# Autodesk Inventor assembly: Cangrejo-Sin-Reductores
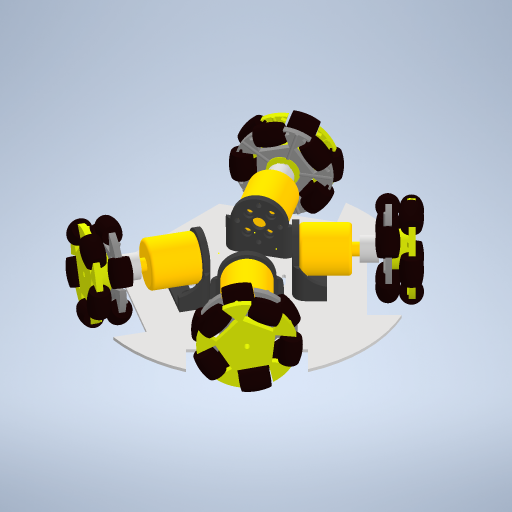
[picture p0: Inventor's stored thumbnail of the model, 512x512]
Saved by Autodesk Inventor 2024 (Build 280153000, 153)
## iProperties
Created: 2023-11-21
Part Number: Cangrejo-Sin-Reductores
Document SubType Name: Assembly
Designer: felip
Author: felip
## Documents named in this file (5)
- C:\Users\felip\Downloads\Gemelo Digital V2\Cangrejo-Sin-Reductores.iam
- C:\Users\felip\Downloads\Gemelo Digital V2\BaseV7.ipt
- C:\Users\felip\Downloads\Gemelo Digital V2\Motor-Soporte-Montaje.iam
- C:\Users\felip\Downloads\Gemelo Digital V2\OMNIWHEELV4.iam
- C:\Users\felip\Downloads\Gemelo Digital V2\Pseudo-SunGear.ipt
## Components (13 placed, 4 different names)
1. BaseV7:1 — Rotational:1, Rotational:2, Rotational:3, Rotational:4, Rotational:12, Rotational:13, Rotational:15, Rotational:16
2. Motor-Soporte-Montaje:1 [sub-assembly] — Rotational:1, Rotational:2, Rotational:7
3. OMNIWHEELV4:1 [sub-assembly] — Rotational:14
4. Pseudo-SunGear:2 — Rotational:7, Rotational:17
5. Pseudo-SunGear:4 — Rotational:8, Rotational:14
6. Motor-Soporte-Montaje:2 [sub-assembly] — Rotational:3, Rotational:4, Rotational:8
7. OMNIWHEELV4:2 [sub-assembly] — Rotational:9
8. OMNIWHEELV4:4 [sub-assembly] — Rotational:17
9. Pseudo-SunGear:5 — Rotational:9
10. Motor-Soporte-Montaje:4 [sub-assembly] — Rotational:15, Rotational:16
11. OMNIWHEELV4:5 [sub-assembly]
12. Pseudo-SunGear:6
13. Motor-Soporte-Montaje:5 [sub-assembly] — Rotational:12, Rotational:13
## Relationships (16: RevoluteJoint 16)
- Rotational:1 [RevoluteJoint]: BaseV7:1 ↔ Motor-Soporte-Montaje:1
- Rotational:2 [RevoluteJoint]: BaseV7:1 ↔ Motor-Soporte-Montaje:1
- Rotational:3 [RevoluteJoint]: BaseV7:1 ↔ Motor-Soporte-Montaje:2
- Rotational:4 [RevoluteJoint]: BaseV7:1 ↔ Motor-Soporte-Montaje:2
- [RevoluteJoint]: Pseudo-SunGear:5 ↔ Motor-Soporte-Montaje:4
- Rotational:7 [RevoluteJoint]: Motor-Soporte-Montaje:1 ↔ Pseudo-SunGear:2
- Rotational:8 [RevoluteJoint]: Pseudo-SunGear:4 ↔ Motor-Soporte-Montaje:2
- Rotational:9 [RevoluteJoint]: OMNIWHEELV4:2 ↔ Pseudo-SunGear:5
- [RevoluteJoint]: Pseudo-SunGear:6 ↔ Motor-Soporte-Montaje:5
- [RevoluteJoint]: OMNIWHEELV4:5 ↔ Pseudo-SunGear:6
- Rotational:12 [RevoluteJoint]: BaseV7:1 ↔ Motor-Soporte-Montaje:5
- Rotational:13 [RevoluteJoint]: BaseV7:1 ↔ Motor-Soporte-Montaje:5
- Rotational:14 [RevoluteJoint]: OMNIWHEELV4:1 ↔ Pseudo-SunGear:4
- Rotational:15 [RevoluteJoint]: BaseV7:1 ↔ Motor-Soporte-Montaje:4
- Rotational:16 [RevoluteJoint]: BaseV7:1 ↔ Motor-Soporte-Montaje:4
- Rotational:17 [RevoluteJoint]: Pseudo-SunGear:2 ↔ OMNIWHEELV4:4
## Named parameters: d10_d8 = 0 mm, d11_d9 = 173.682481 deg, d18_d10_d8 = 0 mm, d19_d11_d9 = 8.424001 deg, d20_d16 = 0 mm, d21_d17 = 17.39851 deg
